# Autodesk Inventor assembly: ESP-WROVER
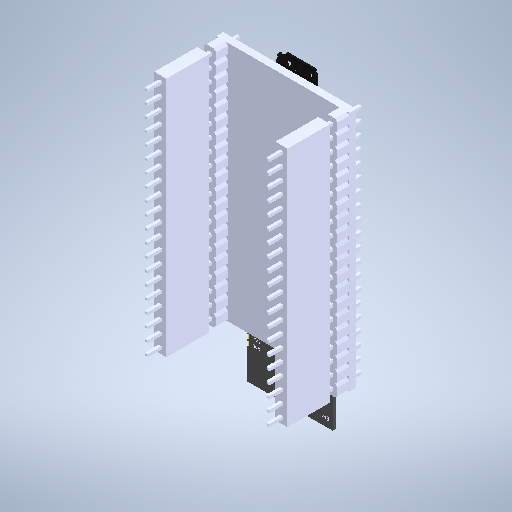
[picture p0: Inventor's stored thumbnail of the model, 512x512]
Saved by Autodesk Inventor 2025.1 (Build 291241020, 241B)
## iProperties
Created: 2025-04-16
Part Number: ESP-WROVER
Document SubType Name: Assembly
Designer: mexen
Author: mexen
## Documents named in this file (3)
- D:\HTL_Anichstrasse\Werkstaette\R6_Drone\Platine_Drohne\Bauteile\ESP32_WROVER\3D\ESP-WROVER.iam
- D:\HTL_Anichstrasse\Werkstaette\R6_Drone\Platine_Drohne\Bauteile\ESP32_WROVER\3D\AB2_USB_MICRO_SMD.ipt
- D:\HTL_Anichstrasse\Werkstaette\R6_Drone\Platine_Drohne\Bauteile\ESP32_WROVER\3D\ESP32-WROVER-Module.ipt
## Components (2 placed, 2 different names)
1. AB2_USB_MICRO_SMD:1 — Passend:1, Fluchtend:1, Fluchtend:2
2. ESP32-WROVER-Module:1 — Passend:1, Fluchtend:1, Fluchtend:2
## Relationships (3: Flush 2, Mate 1)
- Passend:1 [Mate]: AB2_USB_MICRO_SMD:1 ↔ ESP32-WROVER-Module:1
- Fluchtend:1 [Flush]: AB2_USB_MICRO_SMD:1 ↔ ESP32-WROVER-Module:1
- Fluchtend:2 [Flush] (10.24 mm): AB2_USB_MICRO_SMD:1 ↔ ESP32-WROVER-Module:1
